# Autodesk Inventor assembly: Ensamblaje1
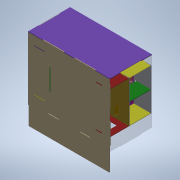
[picture p0: Inventor's stored thumbnail of the model, 180x180]
Saved by Autodesk Inventor 2020 (Build 240168000, 168)
## iProperties
Created: 2020-03-09
Part Number: Ensamblaje1
Material: Genérico
Document SubType Name: Assembly
Designer: joser
Author: joser
## Documents named in this file (16)
- C:\Users\joser\OneDrive\Documentos\UVG\2020\Digital 2\Proyecto\Maqueta\Ensamblaje Total.iam
- C:\Users\joser\OneDrive\Documentos\UVG\2020\Digital 2\Proyecto\Maqueta\Control techo.ipt
- C:\Users\joser\OneDrive\Documentos\UVG\2020\Digital 2\Proyecto\Maqueta\Control Frontal.ipt
- C:\Users\joser\OneDrive\Documentos\UVG\2020\Digital 2\Proyecto\Maqueta\Control lateral.ipt
- C:\Users\joser\OneDrive\Documentos\UVG\2020\Digital 2\Proyecto\Maqueta\Control lateral ventilador.ipt
- C:\Users\joser\OneDrive\Documentos\UVG\2020\Digital 2\Proyecto\Maqueta\Control vidrio.ipt
- C:\Users\joser\OneDrive\Documentos\UVG\2020\Digital 2\Proyecto\Maqueta\Base.ipt
- C:\Users\joser\OneDrive\Documentos\UVG\2020\Digital 2\Proyecto\Maqueta\Base lateral control.ipt
- C:\Users\joser\OneDrive\Documentos\UVG\2020\Digital 2\Proyecto\Maqueta\Base trasera.ipt
- C:\Users\joser\OneDrive\Documentos\UVG\2020\Digital 2\Proyecto\Maqueta\Parte alvaro\Proyecto\Assembly2.iam
- C:\Users\joser\OneDrive\Documentos\UVG\2020\Digital 2\Proyecto\Maqueta\Varilla.ipt
- C:\Users\joser\OneDrive\Documentos\UVG\2020\Digital 2\Proyecto\Maqueta\Parte alvaro\Ensamblaje1.iam
- C:\Users\joser\OneDrive\Documentos\UVG\2020\Digital 2\Proyecto\Maqueta\Parte alvaro\Proyecto\Assembly1.iam
- C:\Users\joser\OneDrive\Documentos\UVG\2020\Digital 2\Proyecto\Maqueta\Celda ensamblaje.iam
- C:\Users\joser\OneDrive\Documentos\UVG\2020\Digital 2\Proyecto\Maqueta\Parte alvaro\Proyecto\Part4.ipt
- C:\Users\joser\OneDrive\Documentos\UVG\2020\Digital 2\Proyecto\Maqueta\Base lateral cafe.ipt
## Components (22 placed, 15 different names)
1. Control techo:1 — Coincidencia:1, Coincidencia:2, Coincidencia:3, Coincidencia:4, Coincidencia:5, Coincidencia:6, Coincidencia:7, Coincidencia:8, Coincidencia:9
2. Control Frontal:1 — Coincidencia:4, Coincidencia:5, Coincidencia:6, Coincidencia:10, Coincidencia:11, Nivelación:1
3. Control lateral:1 — Coincidencia:7, Coincidencia:8, Coincidencia:9, Coincidencia:12, Coincidencia:13, Coincidencia:14
4. Control lateral ventilador:1 — Coincidencia:1, Coincidencia:2, Coincidencia:3
5. Control vidrio:1 — Coincidencia:10, Coincidencia:11, Nivelación:1
6. Base:1 — Coincidencia:12, Coincidencia:13, Coincidencia:14, Coincidencia:21, Coincidencia:22, Coincidencia:23, Coincidencia:24, Coincidencia:25, Coincidencia:26, Coincidencia:27, Coincidencia:30, Nivelación:2, Coincidencia:31, Nivelación:3, Coincidencia:32, Nivelación:4, Coincidencia:33, Nivelación:5, Coincidencia:49, Coincidencia:50, Coincidencia:51
7. Base lateral control:2 — Coincidencia:24, Coincidencia:25, Coincidencia:26, Coincidencia:29
8. Base trasera:1 — Coincidencia:21, Coincidencia:22, Coincidencia:23, Coincidencia:28, Coincidencia:47, Coincidencia:48
9. Assembly2:1 [sub-assembly] — Coincidencia:27, Coincidencia:28, Coincidencia:29, Coincidencia:34, Nivelación:6
10. Varilla:1 — Coincidencia:30, Nivelación:2, Coincidencia:35, Nivelación:7
11. Varilla:2 — Coincidencia:33, Nivelación:5, Coincidencia:38, Nivelación:10
12. Varilla:3 — Coincidencia:31, Nivelación:3, Coincidencia:36, Nivelación:8
13. Varilla:4 — Coincidencia:32, Nivelación:4, Coincidencia:37, Nivelación:9
14. Varilla:5 — Coincidencia:34, Nivelación:6, Coincidencia:44, Nivelación:15
15. Ensamblaje1:1 [sub-assembly] — Coincidencia:36, Nivelación:8, Nivelación:14
16. Ensamblaje1:2 [sub-assembly] — Coincidencia:35, Nivelación:7, Nivelación:13
17. Ensamblaje1:3 [sub-assembly] — Coincidencia:37, Nivelación:9, Nivelación:14
18. Ensamblaje1:4 [sub-assembly] — Coincidencia:38, Nivelación:10, Nivelación:13
19. Assembly1:1 [sub-assembly] — Coincidencia:41, Nivelación:12, Coincidencia:50, Coincidencia:51, Coincidencia:52
20. Celda ensamblaje:1 [sub-assembly] — Coincidencia:41, Nivelación:12, Coincidencia:53
21. Part4:1 — Coincidencia:44, Nivelación:15
22. Base lateral cafe:1 — Coincidencia:47, Coincidencia:48, Coincidencia:49, Coincidencia:52, Coincidencia:53
## Relationships (55: Mate 41, Flush 14)
- Coincidencia:1 [Mate]: Control techo:1 ↔ Control lateral ventilador:1
- Coincidencia:2 [Mate]: Control techo:1 ↔ Control lateral ventilador:1
- Coincidencia:3 [Mate]: Control techo:1 ↔ Control lateral ventilador:1
- Coincidencia:4 [Mate]: Control techo:1 ↔ Control Frontal:1
- Coincidencia:5 [Mate]: Control techo:1 ↔ Control Frontal:1
- Coincidencia:6 [Mate]: Control techo:1 ↔ Control Frontal:1
- Coincidencia:7 [Mate]: Control techo:1 ↔ Control lateral:1
- Coincidencia:8 [Mate]: Control techo:1 ↔ Control lateral:1
- Coincidencia:9 [Mate]: Control techo:1 ↔ Control lateral:1
- Coincidencia:10 [Mate]: Control Frontal:1 ↔ Control vidrio:1
- Coincidencia:11 [Mate]: Control Frontal:1 ↔ Control vidrio:1
- Nivelación:1 [Flush]: Control Frontal:1 ↔ Control vidrio:1
- Coincidencia:12 [Mate]: Control lateral:1 ↔ Base:1
- Coincidencia:13 [Mate]: Control lateral:1 ↔ Base:1
- Coincidencia:14 [Mate]: Control lateral:1 ↔ Base:1
- Coincidencia:21 [Mate]: Base:1 ↔ Base trasera:1
- Coincidencia:22 [Mate]: Base:1 ↔ Base trasera:1
- Coincidencia:23 [Mate]: Base:1 ↔ Base trasera:1
- Coincidencia:24 [Mate]: Base:1 ↔ Base lateral control:2
- Coincidencia:25 [Mate]: Base:1 ↔ Base lateral control:2
- Coincidencia:26 [Mate]: Base:1 ↔ Base lateral control:2
- Coincidencia:27 [Mate]: Base:1 ↔ Assembly2:1
- Coincidencia:28 [Mate]: Base trasera:1 ↔ Assembly2:1
- Coincidencia:29 [Mate] (167 mm): Base lateral control:2 ↔ Assembly2:1
- Coincidencia:30 [Mate]: Base:1 ↔ Varilla:1
- Nivelación:2 [Flush]: Base:1 ↔ Varilla:1
- Coincidencia:31 [Mate]: Base:1 ↔ Varilla:3
- Nivelación:3 [Flush]: Base:1 ↔ Varilla:3
- Coincidencia:32 [Mate]: Base:1 ↔ Varilla:4
- Nivelación:4 [Flush]: Base:1 ↔ Varilla:4
- Coincidencia:33 [Mate]: Base:1 ↔ Varilla:2
- Nivelación:5 [Flush]: Base:1 ↔ Varilla:2
- Coincidencia:34 [Mate]: Assembly2:1 ↔ Varilla:5
- Nivelación:6 [Flush]: Assembly2:1 ↔ Varilla:5
- Coincidencia:35 [Mate]: Varilla:1 ↔ Ensamblaje1:2
- Nivelación:7 [Flush]: Varilla:1 ↔ Ensamblaje1:2
- Coincidencia:36 [Mate]: Varilla:3 ↔ Ensamblaje1:1
- Nivelación:8 [Flush]: Varilla:3 ↔ Ensamblaje1:1
- Coincidencia:37 [Mate]: Varilla:4 ↔ Ensamblaje1:3
- Coincidencia:38 [Mate]: Varilla:2 ↔ Ensamblaje1:4
- Nivelación:9 [Flush]: Varilla:4 ↔ Ensamblaje1:3
- Nivelación:10 [Flush]: Varilla:2 ↔ Ensamblaje1:4
- Coincidencia:41 [Mate]: Assembly1:1 ↔ Celda ensamblaje:1
- Nivelación:12 [Flush]: Assembly1:1 ↔ Celda ensamblaje:1
- Nivelación:13 [Flush]: Ensamblaje1:2 ↔ Ensamblaje1:4
- Nivelación:14 [Flush]: Ensamblaje1:1 ↔ Ensamblaje1:3
- Coincidencia:44 [Mate]: Varilla:5 ↔ Part4:1
- Nivelación:15 [Flush]: Varilla:5 ↔ Part4:1
- Coincidencia:47 [Mate]: Base trasera:1 ↔ Base lateral cafe:1
- Coincidencia:48 [Mate]: Base trasera:1 ↔ Base lateral cafe:1
- Coincidencia:49 [Mate]: Base:1 ↔ Base lateral cafe:1
- Coincidencia:50 [Mate]: Base:1 ↔ Assembly1:1
- Coincidencia:51 [Mate]: Base:1 ↔ Assembly1:1
- Coincidencia:52 [Mate]: Assembly1:1 ↔ Base lateral cafe:1
- Coincidencia:53 [Mate]: Celda ensamblaje:1 ↔ Base lateral cafe:1
